# Autodesk Inventor assembly: SAR330  x 5 + front couplers
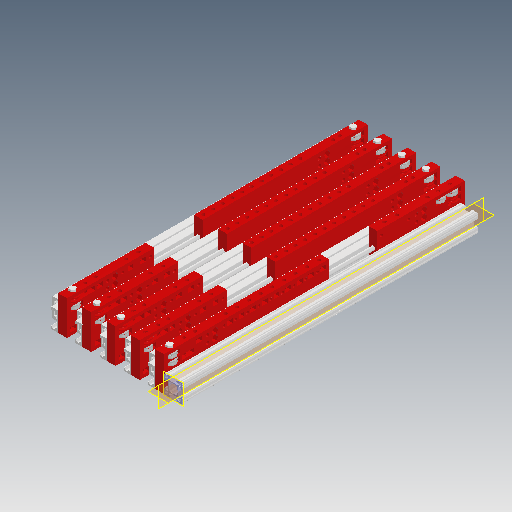
[picture p0: Inventor's stored thumbnail of the model, 512x512]
Saved by Autodesk Inventor 2020 (Build 240168000, 168)
## iProperties
Created: 2019-11-17
Part Number: SAR330  x 5 + front couplers
Document SubType Name: Assembly
Designer: ball
Author: ball
## Documents named in this file (4)
- C:\FTC\FTC8863CAD\2019 Robot\Delivery\SAR330  x 5 + front couplers.iam
- C:\FTC\FTC8863CAD\2019 Robot\Delivery\SAR330 x 4 + regular couplers offset.iam
- C:\FTC\FTC8863CAD\2019 Robot\Delivery\SAR330 + fixed couplers front.iam
- C:\FTC\FTC8863CAD\StepLibraries\Screws\M3 x 20 HEX HEAD CAP SCREW.ipt
## Components (5 placed, 3 different names)
1. SAR330 x 4 + regular couplers offset:1 [sub-assembly] — Mate:1, Mate:2, Mate:3, Mate:4, Mate:5, Mate:6, Mate:8, Mate:9, Mate:10
2. SAR330 + fixed couplers front:1 [sub-assembly] — Mate:1, Mate:2, Mate:3
3. M3 x 20 HEX HEAD CAP SCREW:1 — Mate:4, Mate:8
4. M3 x 20 HEX HEAD CAP SCREW:2 — Mate:5, Mate:9
5. M3 x 20 HEX HEAD CAP SCREW:3 — Mate:6, Mate:10
## Relationships (9: Mate 9)
- Mate:1: SAR330 x 4 + regular couplers offset:1 ↔ SAR330 + fixed couplers front:1
- Mate:2: SAR330 x 4 + regular couplers offset:1 ↔ SAR330 + fixed couplers front:1
- Mate:3: SAR330 x 4 + regular couplers offset:1 ↔ SAR330 + fixed couplers front:1
- Mate:4: SAR330 x 4 + regular couplers offset:1 ↔ M3 x 20 HEX HEAD CAP SCREW:1
- Mate:5: SAR330 x 4 + regular couplers offset:1 ↔ M3 x 20 HEX HEAD CAP SCREW:2
- Mate:6: SAR330 x 4 + regular couplers offset:1 ↔ M3 x 20 HEX HEAD CAP SCREW:3
- Mate:8: SAR330 x 4 + regular couplers offset:1 ↔ M3 x 20 HEX HEAD CAP SCREW:1
- Mate:9: SAR330 x 4 + regular couplers offset:1 ↔ M3 x 20 HEX HEAD CAP SCREW:2
- Mate:10: SAR330 x 4 + regular couplers offset:1 ↔ M3 x 20 HEX HEAD CAP SCREW:3
